# Autodesk Inventor assembly: Mx64_with_bearing_MIR
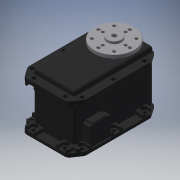
[picture p0: Inventor's stored thumbnail of the model, 180x180]
Saved by Autodesk Inventor 2016 (Build 200138000, 138)
## iProperties
Created: 2014-04-23
Part Number: Mx64_with_bearing_MIR
Document SubType Name: Assembly
Designer: keks
Author: BitBots
## Documents named in this file (4)
- C:\Hambot2\motors\MX64\Mx64_with_bearing_MIR.iam
- C:\Hambot2\motors\MX64\MX64_body_modified_MIR.ipt
- C:\Hambot2\motors\MX64\HN05-i1_MIR.ipt
- C:\Hambot2\motors\MX64\HN05-N101_MIR.ipt
## Components (3 placed, 3 different names)
1. MX64_body_modified_MIR:1 — Mate:1, Flush:2, Flush:1, Rotational:4, Rotational:5
2. HN05-i1_MIR:1 — Rotational:4
3. HN05-N101_MIR:1 — Rotational:5
## Relationships (5: Mate 2, RevoluteJoint 2, Flush 1)
- Mate:1: MX64_body_modified_MIR:1
- Flush:2 [Mate]: MX64_body_modified_MIR:1
- Flush:1: MX64_body_modified_MIR:1
- Rotational:4 [RevoluteJoint]: MX64_body_modified_MIR:1 ↔ HN05-i1_MIR:1
- Rotational:5 [RevoluteJoint]: MX64_body_modified_MIR:1 ↔ HN05-N101_MIR:1
